# Autodesk Inventor assembly: arm
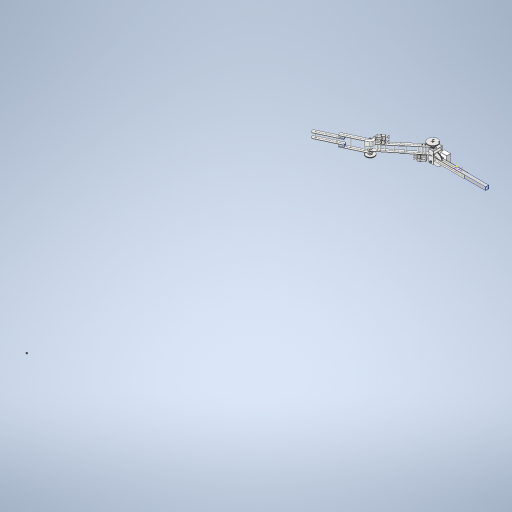
[picture p0: Inventor's stored thumbnail of the model, 512x512]
Saved by Autodesk Inventor 2024 (Build 280153000, 153)
## iProperties
Created: 2025-08-05
Part Number: arm
Document SubType Name: Assembly
Designer: HosodaLab2
Author: HosodaLab2
## iProperties of the stored document CSH-SUS-M6-130.ipt
Created: 2014-02-13
Part Number: CSH-SUS-M6-130
Material: 一般
Document SubType Name: Modeling
Designer: HosodaLab2
Density: 1 g/cm^3
Appearance: 既定
Sending System: SolidWorks 2007
Last Author: guan-li
Last Saved: 2014-03-10
Author: HosodaLab2
## Documents named in this file (52)
- C:\Users\HosodaLab2\OneDrive - Kyoto University\ドキュメント\Inventor\arm\arm.iam
- C:\Users\HosodaLab2\OneDrive - Kyoto University\ドキュメント\Inventor\arm\arm_jig.ipt
- C:\Users\HosodaLab2\OneDrive - Kyoto University\ドキュメント\Inventor\arm\elbow_stopper.ipt
- C:\Users\HosodaLab2\OneDrive - Kyoto University\ドキュメント\Inventor\arm\shoulder2_upper_plate.ipt
- C:\Users\HosodaLab2\OneDrive - Kyoto University\ドキュメント\Inventor\arm\base.ipt
- C:\Users\HosodaLab2\OneDrive - Kyoto University\ドキュメント\Inventor\arm\elbow_lower_plate.ipt
- C:\Users\HosodaLab2\OneDrive - Kyoto University\ドキュメント\Inventor\arm\elbow_upper_plate.ipt
- C:\Users\HosodaLab2\OneDrive - Kyoto University\ドキュメント\Inventor\arm\shoulder_stopper.ipt
- C:\Users\HosodaLab2\OneDrive - Kyoto University\ドキュメント\Inventor\arm\CUI_AMT102-1024-I8000-S.iam
- C:\Users\HosodaLab2\OneDrive - Kyoto University\ドキュメント\Inventor\arm\STHRANG8-MB.iam
- C:\Users\HosodaLab2\OneDrive - Kyoto University\ドキュメント\Inventor\arm\F686ZZ.ipt
- C:\Users\HosodaLab2\OneDrive - Kyoto University\ドキュメント\Inventor\arm\shoulder1_shaft.ipt
- C:\Users\HosodaLab2\OneDrive - Kyoto University\ドキュメント\Inventor\arm\elbow_shaft.ipt
- C:\Users\HosodaLab2\OneDrive - Kyoto University\ドキュメント\Inventor\arm\pully_elbow.ipt
- C:\Users\HosodaLab2\OneDrive - Kyoto University\ドキュメント\Inventor\arm\pully_shoulder1.ipt
- C:\Users\HosodaLab2\OneDrive - Kyoto University\ドキュメント\Inventor\arm\shoulder1_upper_plate.ipt
- C:\Users\HosodaLab2\OneDrive - Kyoto University\ドキュメント\Inventor\arm\shoulder1_shaftholder_spacer_bottom.ipt
- C:\Users\HosodaLab2\OneDrive - Kyoto University\ドキュメント\Inventor\arm\shoulder1_shaftholder_spacer_upper.ipt
- C:\Users\HosodaLab2\OneDrive - Kyoto University\ドキュメント\Inventor\arm\shoulder1_upper_enocder_spacer.ipt
- C:\Users\HosodaLab2\OneDrive - Kyoto University\ドキュメント\Inventor\arm\shoulder1_under_lower_plate_spacer.ipt
- C:\Users\HosodaLab2\OneDrive - Kyoto University\ドキュメント\Inventor\arm\shoulder1_lower_cover.ipt
- C:\Users\HosodaLab2\OneDrive - Kyoto University\ドキュメント\Inventor\arm\shoulder1_upper_cover.ipt
- C:\Users\HosodaLab2\OneDrive - Kyoto University\ドキュメント\Inventor\arm\shoulder1_verticval_left_cover.ipt
- C:\Users\HosodaLab2\OneDrive - Kyoto University\ドキュメント\Inventor\arm\shoulder1_verticval_right_cover.ipt
- C:\Users\HosodaLab2\OneDrive - Kyoto University\ドキュメント\Inventor\arm\STHRANG10-MB_ss.ipt
- C:\Users\HosodaLab2\OneDrive - Kyoto University\ドキュメント\Inventor\arm\shoulder1_lower_plate.ipt
- C:\Users\HosodaLab2\OneDrive - Kyoto University\ドキュメント\Inventor\arm\F688ZZ.iam
- C:\Users\HosodaLab2\OneDrive - Kyoto University\ドキュメント\Inventor\arm\SCST6-8.iam
- C:\Users\HosodaLab2\OneDrive - Kyoto University\ドキュメント\Inventor\arm\shoulder2_upper_plate_spacer.ipt
- C:\Users\HosodaLab2\OneDrive - Kyoto University\ドキュメント\Inventor\arm\shoulder1_encorder_spacer.ipt
- C:\Users\HosodaLab2\OneDrive - Kyoto University\ドキュメント\Inventor\arm\shoulder2_pully_spacer.ipt
- C:\Users\HosodaLab2\OneDrive - Kyoto University\ドキュメント\Inventor\arm\pully_shoulder2.ipt
- pully_shoulder_2_80.ipt
- C:\Users\HosodaLab2\OneDrive - Kyoto University\ドキュメント\Inventor\arm\shoulder2_upperplate_left_spacer.ipt
- C:\Users\HosodaLab2\OneDrive - Kyoto University\ドキュメント\Inventor\arm\shoulder2_upperplate_right_spacer.ipt
- C:\Users\HosodaLab2\OneDrive - Kyoto University\ドキュメント\Inventor\arm\shoulder2_lower_left_plate.ipt
- C:\Users\HosodaLab2\OneDrive - Kyoto University\ドキュメント\Inventor\arm\shoulder2_lower_right_plate.ipt
- C:\Users\HosodaLab2\OneDrive - Kyoto University\ドキュメント\Inventor\arm\elbow_encorder_spacer.ipt
- C:\Users\HosodaLab2\OneDrive - Kyoto University\ドキュメント\Inventor\arm\elbow_upperplate_left_spacer.ipt
- C:\Users\HosodaLab2\OneDrive - Kyoto University\ドキュメント\Inventor\arm\elbow_upperplate_right_spacer.ipt
- C:\Users\HosodaLab2\OneDrive - Kyoto University\ドキュメント\Inventor\arm\elbow_pully_spacer.ipt
- C:\Users\HosodaLab2\OneDrive - Kyoto University\ドキュメント\Inventor\arm\shoulder2_lower_plate_spacer.ipt
- C:\Users\HosodaLab2\OneDrive - Kyoto University\ドキュメント\Inventor\arm\elbow_lower_plate_spacer.ipt
- C:\Users\HosodaLab2\OneDrive - Kyoto University\ドキュメント\Inventor\arm\elbow_upper_plate_spacer.ipt
- C:\Users\HosodaLab2\OneDrive - Kyoto University\ドキュメント\Inventor\arm\shoulder1_NewPart2.ipt
- **C:\Users\HosodaLab2\OneDrive - Kyoto University\ドキュメント\Inventor\arm\arm.iam*LocalDocs*xAaaaalcaAaaaaaaaAaaaqn4oUb*CSH-SUS-M6-130.ipt
- C:\Users\HosodaLab2\OneDrive - Kyoto University\ドキュメント\Inventor\arm\shoulder2_elbow_strain_sensor_near.iam
- C:\Users\HosodaLab2\OneDrive - Kyoto University\ドキュメント\Inventor\arm\shoulder2_elbow_strain_sensor_away.iam
- C:\Users\HosodaLab2\OneDrive - Kyoto University\ドキュメント\Inventor\arm\shoulder1_uppper_plate_bolt_spcaer.ipt
- C:\Users\HosodaLab2\OneDrive - Kyoto University\ドキュメント\Inventor\arm\shoulder1_lower_plate_bolt_spcaer.ipt
- C:\Users\HosodaLab2\OneDrive - Kyoto University\ドキュメント\Inventor\arm\shoulder2_shaft2.ipt
- C:\Users\HosodaLab2\OneDrive - Kyoto University\ドキュメント\Inventor\arm\CSH-SUS-M6-130.SLDPRT
## Components (76 placed, 49 different names)
1. arm_jig:1 — 回転:140, 回転:141, 回転:142, 回転:143
2. base:1 — 回転:33, 回転:34, 回転:73, 回転:74
3. elbow_lower_plate:1 — 回転:142, 回転:143, リジッド:2, 回転:167
4. elbow_stopper:1 — 回転:168, 回転:169
5. shoulder1_encorder_spacer:1 — 回転:62, 回転:63
6. shoulder_stopper:1 — 回転:58, 回転:59
7. shoulder1_plate:1 — 回転:33, 回転:34, 角度:3, 回転:58, 回転:59, 回転:62, 回転:63, 回転:89, 角度:5
8. elbow_upper_plate:2 — 回転:140, 回転:141, 回転:144, 回転:148, 回転:149, 回転:153
9. shoulder2_lower_left_plate:1 — 回転:132, 回転:133, 角度:9, 回転:152, 回転:182, 回転:183, 回転:184, 回転:185
10. shoulder2_upper_plate:2 — メイト:1, 回転:127, 回転:128, 回転:173, 回転:175, メイト:3, 回転:184, 回転:185, 回転:197
11. shoulder2_lower_right_plate:1 — 回転:106, 回転:151, 回転:168, 回転:169, メイト:5, 回転:186, 回転:187, 回転:190, 回転:191
12. shoulder2_upper_plate:3 — 回転:122, 回転:130, 回転:186, 回転:187, 回転:198, 回転:200, 回転:201, 回転:202, 回転:203, 回転:204
13. arm_jig:2
14. elbow_lower_plate:3 — 回転:155, 回転:156
15. elbow_upper_plate:3 — 回転:154, 回転:161, 回転:162, 回転:163, 回転:166, リジッド:1
16. CUI_AMT102-1024-I8000-S:1 [sub-assembly] — 回転:194, 回転:199
17. CUI_AMT102-1024-I8000-S:3 [sub-assembly] — 角度:3, 回転:87, 回転:92
18. F686ZZ:1
19. pully_elbow:1 — 回転:164, 回転:165
20. pully_shoulder1:3 — 回転:157, 回転:158
21. shoulder1_shaftholder_spacer_bottom:1 — 回転:79, 回転:121
22. shoulder1_shaftholder_spacer_upper:1 — 回転:83
23. shoulder1_upper_enocder_spacer:1 — 回転:87, 回転:95, 回転:96
24. shoulder1_under_lower_plate_spacer:1 — 回転:93, 回転:109
25. shoulder1_upper_cover:1 — 角度:5, 回転:95, 回転:96, 回転:98, 回転:99, 回転:207, 回転:208, 回転:209, 回転:210
26. shoulder1_verticval_right_cover:1 — 回転:193, 回転:194, 回転:209, 回転:210
27. shoulder1_verticval_left_cover:1 — 回転:192, 回転:196, 回転:207, 回転:208
28. STHRANG10-MB_ss:1 — 回転:79, 回転:83, 回転:157, 回転:158
29. STHRANG8-MB:2 [sub-assembly] — 回転:123, 回転:124, 円柱状:8, 回転:159
30. shoulder1_lower_plate:1 — 回転:73, 回転:74, 回転:88, 角度:7
31. F688ZZ:1 [sub-assembly] — 回転:88, 回転:93, 回転:121, 回転:211
32. F688ZZ:2 [sub-assembly] — 回転:89, 回転:92
33. SCST6-8:1 [sub-assembly] — 回転:98, 回転:99
34. SCST6-8:2 [sub-assembly] — 回転:205, 回転:206
35. shoulder2_upper_plate_spacer:1 — 回転:173, 回転:200
36. F688ZZ:3 [sub-assembly] — 回転:106, 回転:137
37. F688ZZ:4 [sub-assembly] — 回転:134, 回転:212
38. shoulder1_lower_cover:2 — 角度:7, 回転:109, メイト:1, 回転:205, 回転:206
39. F688ZZ:5 [sub-assembly] — 回転:193
40. F688ZZ:6 [sub-assembly] — 回転:192, 回転:213
41. shoulder1_shaftholder_spacer_bottom:2
42. shoulder2_pully_spacer:1 — 回転:122, 回転:123, 回転:124, 回転:198
43. pully_shoulder_2_80:1 — 円柱状:8, 回転:159
44. STHRANG8-MB:3 [sub-assembly] — 回転:127, 回転:128
45. shoulder2_upperplate_left_spacer:1 — 回転:196, 回転:197
46. shoulder2_upperplate_right_spacer:1 — 回転:130, 回転:199
47. CUI_AMT102-1024-I8000-S:4 [sub-assembly] — 回転:134, 角度:9, 回転:136
48. elbow_encorder_spacer:1 — 回転:132, 回転:133
49. elbow_upperplate_right_spacer:1 — 回転:137, 回転:144
50. elbow_upperplate_left_spacer:2 — 回転:136, 回転:162
51. elbow_pully_spacer:1 — 回転:146, 回転:147, 回転:161, 回転:163
52. STHRANG8-MB:4 [sub-assembly] — 回転:146, 回転:147, 回転:164, 回転:165
53. STHRANG8-MB:5 [sub-assembly] — 回転:148, 回転:149
54. shoulder2_upper_plate_spacer:2 — 回転:175
55. shoulder2_lower_plate_spacer:1 — 回転:151
56. shoulder2_lower_plate_spacer:2 — 回転:152
57. elbow_lower_plate_spacer:1 — 回転:155, リジッド:2
58. elbow_upper_plate_spacer:1 — 回転:153, 回転:166
59. elbow_upper_plate_spacer:2 — 回転:154, リジッド:1
60. elbow_lower_plate_spacer:2 — 回転:156, 回転:167
61. shoulder1_NewPart2:1
62. shoulder2_elbow_strain_sensor_near:1 [sub-assembly] — メイト:3, メイト:4, 円柱状:17, 円柱状:18
63. CSH-SUS-M6-130:1 — 回転:202, 円柱状:18, 円柱状:20
64. CSH-SUS-M6-130:2 — 回転:201, 円柱状:17, 円柱状:19
65. CSH-SUS-M6-130:3 — 回転:183, 円柱状:14, 円柱状:16
66. CSH-SUS-M6-130:4 — 回転:182, 円柱状:13, 円柱状:15
67. shoulder2_elbow_strain_sensor_away:1 [sub-assembly] — メイト:4, 円柱状:19, 円柱状:20
68. shoulder2_elbow_strain_sensor_away:2 [sub-assembly] — 円柱状:15, 円柱状:16, メイト:6
69. shoulder2_elbow_strain_sensor_near:2 [sub-assembly] — 円柱状:13, 円柱状:14, メイト:5, メイト:6
70. shoulder1_uppper_plate_bolt_spcaer:1 — 回転:203
71. shoulder1_uppper_plate_bolt_spcaer:2 — 回転:204
72. shoulder1_lower_plate_bolt_spcaer:1 — 回転:190
73. shoulder1_lower_plate_bolt_spcaer:2 — 回転:191
74. shoulder1_shaft:1 — 回転:211
75. elbow_shaft:1 — 回転:212
76. shoulder2_shaft2:1 — 回転:213
## Relationships (115: RevoluteJoint 95, CylindricalJoint 9, Mate 5, Angle 4, WeldJoint 2)
- [RevoluteJoint]: arm_jig:2 ↔ elbow_upper_plate:3
- [RevoluteJoint]: arm_jig:2 ↔ elbow_upper_plate:3
- [RevoluteJoint]: arm_jig:2 ↔ elbow_lower_plate:3
- [RevoluteJoint]: arm_jig:2 ↔ elbow_lower_plate:3
- 回転:33 [RevoluteJoint]: base:1 ↔ shoulder1_plate:1
- 回転:34 [RevoluteJoint]: base:1 ↔ shoulder1_plate:1
- 角度:3 [Angle] (180 deg): shoulder1_plate:1 ↔ CUI_AMT102-1024-I8000-S:3
- 回転:58 [RevoluteJoint]: shoulder_stopper:1 ↔ shoulder1_plate:1
- 回転:59 [RevoluteJoint]: shoulder_stopper:1 ↔ shoulder1_plate:1
- 回転:62 [RevoluteJoint]: shoulder1_encorder_spacer:1 ↔ shoulder1_plate:1
- 回転:63 [RevoluteJoint]: shoulder1_encorder_spacer:1 ↔ shoulder1_plate:1
- 回転:73 [RevoluteJoint]: base:1 ↔ shoulder1_lower_plate:1
- 回転:74 [RevoluteJoint]: base:1 ↔ shoulder1_lower_plate:1
- 回転:79 [RevoluteJoint]: shoulder1_shaftholder_spacer_bottom:1 ↔ STHRANG10-MB_ss:1
- 回転:83 [RevoluteJoint]: shoulder1_shaftholder_spacer_upper:1 ↔ STHRANG10-MB_ss:1
- 回転:87 [RevoluteJoint]: CUI_AMT102-1024-I8000-S:3 ↔ shoulder1_upper_enocder_spacer:1
- 回転:88 [RevoluteJoint]: shoulder1_lower_plate:1 ↔ F688ZZ:1
- 回転:89 [RevoluteJoint]: shoulder1_plate:1 ↔ F688ZZ:2
- 角度:5 [Angle] (0 deg): shoulder1_plate:1 ↔ shoulder1_upper_cover:1
- 回転:92 [RevoluteJoint]: CUI_AMT102-1024-I8000-S:3 ↔ F688ZZ:2
- 回転:93 [RevoluteJoint]: shoulder1_under_lower_plate_spacer:1 ↔ F688ZZ:1
- 回転:95 [RevoluteJoint]: shoulder1_upper_enocder_spacer:1 ↔ shoulder1_upper_cover:1
- 回転:96 [RevoluteJoint]: shoulder1_upper_enocder_spacer:1 ↔ shoulder1_upper_cover:1
- 回転:98 [RevoluteJoint]: shoulder1_upper_cover:1 ↔ SCST6-8:1
- 回転:99 [RevoluteJoint]: shoulder1_upper_cover:1 ↔ SCST6-8:1
- 回転:106 [RevoluteJoint]: shoulder2_lower_right_plate:1 ↔ F688ZZ:3
- 角度:7 [Angle] (180 deg): shoulder1_lower_plate:1 ↔ shoulder1_lower_cover:2
- 回転:109 [RevoluteJoint]: shoulder1_under_lower_plate_spacer:1 ↔ shoulder1_lower_cover:2
- メイト:1 [Mate] (2.5 mm): shoulder2_upper_plate:2 ↔ shoulder1_lower_cover:2
- 回転:121 [RevoluteJoint]: shoulder1_shaftholder_spacer_bottom:1 ↔ F688ZZ:1
- 回転:122 [RevoluteJoint]: shoulder2_upper_plate:3 ↔ shoulder2_pully_spacer:1
- 回転:123 [RevoluteJoint]: STHRANG8-MB:2 ↔ shoulder2_pully_spacer:1
- 回転:124 [RevoluteJoint]: STHRANG8-MB:2 ↔ shoulder2_pully_spacer:1
- 回転:127 [RevoluteJoint]: shoulder2_upper_plate:2 ↔ STHRANG8-MB:3
- 回転:128 [RevoluteJoint]: shoulder2_upper_plate:2 ↔ STHRANG8-MB:3
- 回転:130 [RevoluteJoint]: shoulder2_upper_plate:3 ↔ shoulder2_upperplate_right_spacer:1
- 回転:132 [RevoluteJoint]: shoulder2_lower_left_plate:1 ↔ elbow_encorder_spacer:1
- 回転:133 [RevoluteJoint]: shoulder2_lower_left_plate:1 ↔ elbow_encorder_spacer:1
- 回転:134 [RevoluteJoint]: F688ZZ:4 ↔ CUI_AMT102-1024-I8000-S:4
- 角度:9 [Angle] (0 deg): shoulder2_lower_left_plate:1 ↔ CUI_AMT102-1024-I8000-S:4
- 回転:136 [RevoluteJoint]: CUI_AMT102-1024-I8000-S:4 ↔ elbow_upperplate_left_spacer:2
- 回転:137 [RevoluteJoint]: F688ZZ:3 ↔ elbow_upperplate_right_spacer:1
- 回転:140 [RevoluteJoint]: arm_jig:1 ↔ elbow_upper_plate:2
- 回転:141 [RevoluteJoint]: arm_jig:1 ↔ elbow_upper_plate:2
- 回転:142 [RevoluteJoint]: arm_jig:1 ↔ elbow_lower_plate:1
- 回転:143 [RevoluteJoint]: arm_jig:1 ↔ elbow_lower_plate:1
- 回転:144 [RevoluteJoint]: elbow_upper_plate:2 ↔ elbow_upperplate_right_spacer:1
- 回転:146 [RevoluteJoint]: elbow_pully_spacer:1 ↔ STHRANG8-MB:4
- 回転:147 [RevoluteJoint]: elbow_pully_spacer:1 ↔ STHRANG8-MB:4
- 回転:148 [RevoluteJoint]: elbow_upper_plate:2 ↔ STHRANG8-MB:5
- 回転:149 [RevoluteJoint]: elbow_upper_plate:2 ↔ STHRANG8-MB:5
- 回転:151 [RevoluteJoint]: shoulder2_lower_right_plate:1 ↔ shoulder2_lower_plate_spacer:1
- 回転:152 [RevoluteJoint]: shoulder2_lower_left_plate:1 ↔ shoulder2_lower_plate_spacer:2
- 回転:153 [RevoluteJoint]: elbow_upper_plate:2 ↔ elbow_upper_plate_spacer:1
- 回転:154 [RevoluteJoint]: elbow_upper_plate:3 ↔ elbow_upper_plate_spacer:2
- 回転:155 [RevoluteJoint]: elbow_lower_plate:3 ↔ elbow_lower_plate_spacer:1
- 回転:156 [RevoluteJoint]: elbow_lower_plate:3 ↔ elbow_lower_plate_spacer:2
- 回転:157 [RevoluteJoint]: pully_shoulder1:3 ↔ STHRANG10-MB_ss:1
- 回転:158 [RevoluteJoint]: pully_shoulder1:3 ↔ STHRANG10-MB_ss:1
- 円柱状:8 [CylindricalJoint]: STHRANG8-MB:2 ↔ pully_shoulder_2_80:1
- 回転:159 [RevoluteJoint]: STHRANG8-MB:2 ↔ pully_shoulder_2_80:1
- 回転:161 [RevoluteJoint]: elbow_upper_plate:3 ↔ elbow_pully_spacer:1
- 回転:162 [RevoluteJoint]: elbow_upper_plate:3 ↔ elbow_upperplate_left_spacer:2
- 回転:163 [RevoluteJoint]: elbow_upper_plate:3 ↔ elbow_pully_spacer:1
- 回転:164 [RevoluteJoint]: pully_elbow:1 ↔ STHRANG8-MB:4
- 回転:165 [RevoluteJoint]: pully_elbow:1 ↔ STHRANG8-MB:4
- 回転:166 [RevoluteJoint]: elbow_upper_plate:3 ↔ elbow_upper_plate_spacer:1
- リジッド:1 [WeldJoint]: elbow_upper_plate:3 ↔ elbow_upper_plate_spacer:2
- リジッド:2 [WeldJoint]: elbow_lower_plate:1 ↔ elbow_lower_plate_spacer:1
- 回転:167 [RevoluteJoint]: elbow_lower_plate:1 ↔ elbow_lower_plate_spacer:2
- 回転:168 [RevoluteJoint]: elbow_stopper:1 ↔ shoulder2_lower_right_plate:1
- 回転:169 [RevoluteJoint]: elbow_stopper:1 ↔ shoulder2_lower_right_plate:1
- 回転:173 [RevoluteJoint]: shoulder2_upper_plate:2 ↔ shoulder2_upper_plate_spacer:1
- 回転:175 [RevoluteJoint]: shoulder2_upper_plate:2 ↔ shoulder2_upper_plate_spacer:2
- 回転:182 [RevoluteJoint]: shoulder2_lower_left_plate:1 ↔ CSH-SUS-M6-130:4
- 回転:183 [RevoluteJoint]: shoulder2_lower_left_plate:1 ↔ CSH-SUS-M6-130:3
- メイト:3 [Mate] (3 mm): shoulder2_upper_plate:2 ↔ shoulder2_elbow_strain_sensor_near:1
- メイト:4 [Mate]: shoulder2_elbow_strain_sensor_near:1 ↔ shoulder2_elbow_strain_sensor_away:1
- 円柱状:13 [CylindricalJoint]: CSH-SUS-M6-130:4 ↔ shoulder2_elbow_strain_sensor_near:2
- 円柱状:14 [CylindricalJoint]: CSH-SUS-M6-130:3 ↔ shoulder2_elbow_strain_sensor_near:2
- メイト:5 [Mate] (3 mm): shoulder2_lower_right_plate:1 ↔ shoulder2_elbow_strain_sensor_near:2
- 円柱状:15 [CylindricalJoint]: CSH-SUS-M6-130:4 ↔ shoulder2_elbow_strain_sensor_away:2
- 円柱状:16 [CylindricalJoint]: CSH-SUS-M6-130:3 ↔ shoulder2_elbow_strain_sensor_away:2
- メイト:6 [Mate]: shoulder2_elbow_strain_sensor_away:2 ↔ shoulder2_elbow_strain_sensor_near:2
- 回転:184 [RevoluteJoint]: shoulder2_lower_left_plate:1 ↔ shoulder2_upper_plate:2
- 回転:185 [RevoluteJoint]: shoulder2_lower_left_plate:1 ↔ shoulder2_upper_plate:2
- 回転:186 [RevoluteJoint]: shoulder2_lower_right_plate:1 ↔ shoulder2_upper_plate:3
- 回転:187 [RevoluteJoint]: shoulder2_lower_right_plate:1 ↔ shoulder2_upper_plate:3
- 回転:190 [RevoluteJoint]: shoulder2_lower_right_plate:1 ↔ shoulder1_lower_plate_bolt_spcaer:1
- 回転:191 [RevoluteJoint]: shoulder2_lower_right_plate:1 ↔ shoulder1_lower_plate_bolt_spcaer:2
- 回転:192 [RevoluteJoint]: shoulder1_verticval_left_cover:1 ↔ F688ZZ:6
- 回転:193 [RevoluteJoint]: shoulder1_verticval_right_cover:1 ↔ F688ZZ:5
- 回転:194 [RevoluteJoint]: CUI_AMT102-1024-I8000-S:1 ↔ shoulder1_verticval_right_cover:1
- 回転:196 [RevoluteJoint]: shoulder1_verticval_left_cover:1 ↔ shoulder2_upperplate_left_spacer:1
- 回転:197 [RevoluteJoint]: shoulder2_upper_plate:2 ↔ shoulder2_upperplate_left_spacer:1
- 回転:198 [RevoluteJoint]: shoulder2_upper_plate:3 ↔ shoulder2_pully_spacer:1
- 回転:199 [RevoluteJoint]: CUI_AMT102-1024-I8000-S:1 ↔ shoulder2_upperplate_right_spacer:1
- 回転:200 [RevoluteJoint]: shoulder2_upper_plate:3 ↔ shoulder2_upper_plate_spacer:1
- 回転:201 [RevoluteJoint]: shoulder2_upper_plate:3 ↔ CSH-SUS-M6-130:2
- 回転:202 [RevoluteJoint]: shoulder2_upper_plate:3 ↔ CSH-SUS-M6-130:1
- 円柱状:17 [CylindricalJoint]: shoulder2_elbow_strain_sensor_near:1 ↔ CSH-SUS-M6-130:2
- 円柱状:18 [CylindricalJoint]: shoulder2_elbow_strain_sensor_near:1 ↔ CSH-SUS-M6-130:1
- 円柱状:19 [CylindricalJoint]: CSH-SUS-M6-130:2 ↔ shoulder2_elbow_strain_sensor_away:1
- 円柱状:20 [CylindricalJoint]: CSH-SUS-M6-130:1 ↔ shoulder2_elbow_strain_sensor_away:1
- 回転:203 [RevoluteJoint]: shoulder2_upper_plate:3 ↔ shoulder1_uppper_plate_bolt_spcaer:1
- 回転:204 [RevoluteJoint]: shoulder2_upper_plate:3 ↔ shoulder1_uppper_plate_bolt_spcaer:2
- 回転:205 [RevoluteJoint]: SCST6-8:2 ↔ shoulder1_lower_cover:2
- 回転:206 [RevoluteJoint]: SCST6-8:2 ↔ shoulder1_lower_cover:2
- 回転:207 [RevoluteJoint]: shoulder1_upper_cover:1 ↔ shoulder1_verticval_left_cover:1
- 回転:208 [RevoluteJoint]: shoulder1_upper_cover:1 ↔ shoulder1_verticval_left_cover:1
- 回転:209 [RevoluteJoint]: shoulder1_upper_cover:1 ↔ shoulder1_verticval_right_cover:1
- 回転:210 [RevoluteJoint]: shoulder1_upper_cover:1 ↔ shoulder1_verticval_right_cover:1
- 回転:211 [RevoluteJoint]: F688ZZ:1 ↔ shoulder1_shaft:1
- 回転:212 [RevoluteJoint]: F688ZZ:4 ↔ elbow_shaft:1
- 回転:213 [RevoluteJoint]: F688ZZ:6 ↔ shoulder2_shaft2:1
## Named parameters: d38_d30 = 0 mm, d39_d31 = 90 deg, d40_d32 = 0 mm, d41_d33 = 90 deg, d42_d34 = 0 mm, d43_d35 = 180 deg, d44_d36 = 0 mm, d45_d37 = -90 deg
